# Autodesk Inventor assembly: Leg_Loadpipe_Connector
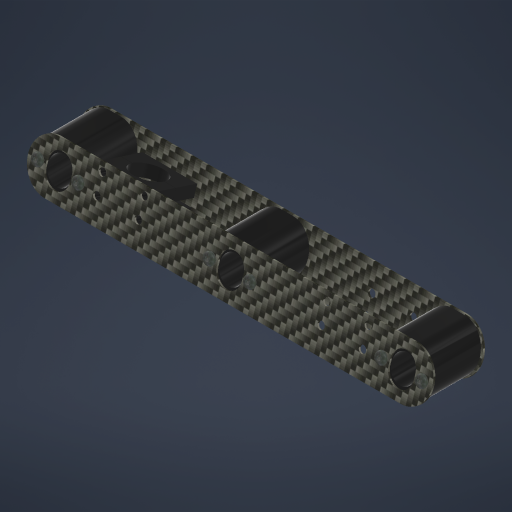
[picture p0: Inventor's stored thumbnail of the model, 512x512]
Saved by Autodesk Inventor 2024 (Build 280153000, 153)
## iProperties
Created: 2023-06-08
Part Number: Leg_Loadpipe_Connector
Document SubType Name: Assembly
Designer: dzw04
Author: dzw04
## Documents named in this file (6)
- C:\Users\dzw04\Saxion\Mechatronica Lectoraat LMECH LED - Database ARG\Component_Database\SAR\01. CAD\01. 3D_Drawing\02. Sub_Assemblies\Leg_Loadpipe_Connector.iam
- C:\Users\dzw04\Saxion\Mechatronica Lectoraat LMECH LED - Database ARG\Component_Database\SAR\01. CAD\01. 3D_Drawing\01. Parts\Leg_Loadpipe_Plate_Inner.ipt
- C:\Users\dzw04\Saxion\Mechatronica Lectoraat LMECH LED - Database ARG\Component_Database\SAR\01. CAD\01. 3D_Drawing\01. Parts\Leg_Loadpipe_Mount.iam
- C:\Users\dzw04\OneDrive - Saxion\Documenten\Inventor\Content Center Files\R2024\en-US\ISO 7380-1\ISO 7380-1 - M3 x 6.ipt
- C:\Users\dzw04\Saxion\Mechatronica Lectoraat LMECH LED - Database ARG\Component_Database\SAR\01. CAD\01. 3D_Drawing\01. Parts\Leg_Loadpipe_Plate_Outer.ipt
- C:\Users\dzw04\Saxion\Mechatronica Lectoraat LMECH LED - Database ARG\Component_Database\SAR\01. CAD\01. 3D_Drawing\01. Parts\16mm_Tube_Connecotor_Holybro.ipt
## Components (21 placed, 5 different names)
1. Leg_Loadpipe_Plate_Inner:1 — Mate:2, Mate:3, Mate:4, Mate:5, Insert:1, Insert:2, Mate:9, Mate:10, Mate:11, Mate:13, Mate:14, Mate:15
2. Leg_Loadpipe_Plate_Outer:1 — Mate:5, Mate:6, Mate:7, Insert:3, Insert:4
3. 16mm_Tube_Connecotor_Holybro:1 — Mate:8, Flush:1, Flush:2, Mate:9, Mate:10, Mate:11
4. 16mm_Tube_Connecotor_Holybro:2 — Mate:8, Flush:1, Flush:2
5. 16mm_Tube_Connecotor_Holybro:3 — Mate:13, Mate:14, Mate:15
6. 16mm_Tube_Connecotor_Holybro:4
7. ISO 7380-1 M3 x 6:1 — Insert:1
8. ISO 7380-1 M3 x 6:2 — Insert:2
9. ISO 7380-1 M3 x 6:3 — Insert:3
10. ISO 7380-1 M3 x 6:4 — Insert:4
11. Leg_Loadpipe_Mount:1 [sub-assembly] — Mate:2, Mate:3, Mate:4, Mate:6, Mate:7
12. ISO 7380-1 M3 x 6:5
13. ISO 7380-1 M3 x 6:6
14. ISO 7380-1 M3 x 6:7
15. ISO 7380-1 M3 x 6:8
16. Leg_Loadpipe_Mount:2 [sub-assembly]
17. ISO 7380-1 M3 x 6:9
18. ISO 7380-1 M3 x 6:10
19. ISO 7380-1 M3 x 6:11
20. ISO 7380-1 M3 x 6:12
21. Leg_Loadpipe_Mount:3 [sub-assembly]
## Component patterns: (3 elements, first: ISO 7380-1 M3 x 6:1 + ISO 7380-1 M3 x 6:2 + ISO 7380-1 M3 x 6:3 + ISO 7380-1 M3 x 6:4 + Leg_Loadpipe_Mount:1)
## Relationships (22: Mate 14, Insert 4, Flush 4)
- Mate:2: Leg_Loadpipe_Plate_Inner:1 ↔ Leg_Loadpipe_Mount:1
- Mate:3: Leg_Loadpipe_Plate_Inner:1 ↔ Leg_Loadpipe_Mount:1
- Mate:4: Leg_Loadpipe_Plate_Inner:1 ↔ Leg_Loadpipe_Mount:1
- Mate:5 (22.5 mm): Leg_Loadpipe_Plate_Inner:1 ↔ Leg_Loadpipe_Plate_Outer:1
- Mate:6: Leg_Loadpipe_Plate_Outer:1 ↔ Leg_Loadpipe_Mount:1
- Mate:7: Leg_Loadpipe_Plate_Outer:1 ↔ Leg_Loadpipe_Mount:1
- Insert:1: Leg_Loadpipe_Plate_Inner:1 ↔ ISO 7380-1 M3 x 6:1
- Insert:2: Leg_Loadpipe_Plate_Inner:1 ↔ ISO 7380-1 M3 x 6:2
- Insert:3: Leg_Loadpipe_Plate_Outer:1 ↔ ISO 7380-1 M3 x 6:3
- Insert:4: Leg_Loadpipe_Plate_Outer:1 ↔ ISO 7380-1 M3 x 6:4
- Mate:8: 16mm_Tube_Connecotor_Holybro:1 ↔ 16mm_Tube_Connecotor_Holybro:2
- Flush:1: 16mm_Tube_Connecotor_Holybro:1 ↔ 16mm_Tube_Connecotor_Holybro:2
- Flush:2: 16mm_Tube_Connecotor_Holybro:1 ↔ 16mm_Tube_Connecotor_Holybro:2
- Mate:9: Leg_Loadpipe_Plate_Inner:1 ↔ 16mm_Tube_Connecotor_Holybro:1
- Mate:10: Leg_Loadpipe_Plate_Inner:1 ↔ 16mm_Tube_Connecotor_Holybro:1
- Mate:11: Leg_Loadpipe_Plate_Inner:1 ↔ 16mm_Tube_Connecotor_Holybro:1
- [Mate]: 16mm_Tube_Connecotor_Holybro:3 ↔ 16mm_Tube_Connecotor_Holybro:4
- [Flush]: 16mm_Tube_Connecotor_Holybro:3 ↔ 16mm_Tube_Connecotor_Holybro:4
- [Flush]: 16mm_Tube_Connecotor_Holybro:3 ↔ 16mm_Tube_Connecotor_Holybro:4
- Mate:13: Leg_Loadpipe_Plate_Inner:1 ↔ 16mm_Tube_Connecotor_Holybro:3
- Mate:14: Leg_Loadpipe_Plate_Inner:1 ↔ 16mm_Tube_Connecotor_Holybro:3
- Mate:15: Leg_Loadpipe_Plate_Inner:1 ↔ 16mm_Tube_Connecotor_Holybro:3
## Named parameters: d95_d90 = 0 mm, d96_d91 = 0 mm, d97_d89 = 0 mm
